# Autodesk Inventor assembly: Zusammenbau
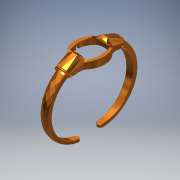
[picture p0: Inventor's stored thumbnail of the model, 180x180]
Saved by Autodesk Inventor 2019 (Build 230136000, 136)
## iProperties
Created: 2021-03-09
Part Number: Zusammenbau
Material: Generisch
Document SubType Name: Assembly
Designer: Bergi
Author: Bergi
## Documents named in this file (4)
- C:\Users\Bergi\Desktop\3D Sketches\Bulova\Zusammenbau.iam
- C:\Users\Bergi\Desktop\3D Sketches\Bulova\Main_afterRhino.ipt
- C:\Users\Bergi\Desktop\3D Sketches\Bulova\bild.ipt
- C:\Users\Bergi\Desktop\3D Sketches\Bulova\Armband_afterrhino.ipt
## Components (4 placed, 3 different names)
1. Main_afterRhino:1 — Fluchtend:1, Passend:3, Passend:4
2. Armband_afterrhino:1 — Passend:3
3. Armband_afterrhino:2 — Passend:4
4. bild:1
## Relationships (5: Flush 3, Mate 2)
- Fluchtend:1 [Flush]: Main_afterRhino:1
- [Flush]: Main_afterRhino:1 ↔ Armband_afterrhino:1
- [Flush]: Main_afterRhino:1 ↔ Armband_afterrhino:2
- Passend:3 [Mate]: Main_afterRhino:1 ↔ Armband_afterrhino:1
- Passend:4 [Mate]: Main_afterRhino:1 ↔ Armband_afterrhino:2
